# Autodesk Inventor assembly: Stange
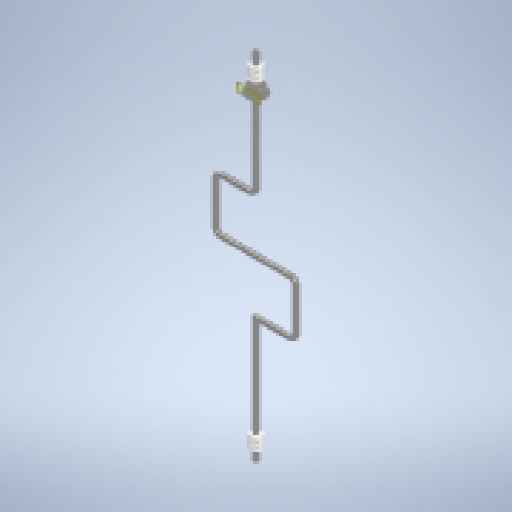
[picture p0: Inventor's stored thumbnail of the model, 512x512]
Saved by Autodesk Inventor 2024.4 (Build 284460000, 460)
## iProperties
Created: 2026-01-10
Part Number: Stange
Description: Stange
Document SubType Name: Assembly
Designer: Philf
Mass: 4853.9 g
Surface Area: 1441.51 cm^2
Volume: 679.011 cm^3
Density: 7.14849 g/cm^3
Masse[kg]: 4,854 kg
## Documents named in this file (3)
- C:\Users\Philf\Documents\Vault\Daten\I60-Konstruktion\I60-Gruppe-7\Tritt\Stange.iam
- C:\Users\Philf\Documents\Vault\Daten\I60-Konstruktion\I60-Gruppe-7\Tritt\Trittstange.ipt
- C:\Users\Philf\Documents\Vault\Daten\I60-Konstruktion\I60-Gruppe-7\Tritt\Stopper.ipt
## Components (3 placed, 2 different names)
1. Trittstange:1 — Passend:7, Passend:8, Fluchtend:5, Fluchtend:6
2. Stopper:2 — Passend:7, Fluchtend:6
3. Stopper:3 — Passend:8, Fluchtend:5
## Relationships (4: Mate 2, Flush 2)
- Passend:7 [Mate]: Trittstange:1 ↔ Stopper:2
- Passend:8 [Mate]: Trittstange:1 ↔ Stopper:3
- Fluchtend:5 [Flush] (40 mm): Trittstange:1 ↔ Stopper:3
- Fluchtend:6 [Flush] (40 mm): Trittstange:1 ↔ Stopper:2
